# Autodesk Inventor assembly: supports
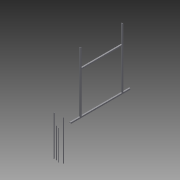
[picture p0: Inventor's stored thumbnail of the model, 180x180]
Saved by Autodesk Inventor 2013 (Build 170138000, 138)
## iProperties
Created: 2012-10-21
Part Number: supports
Document SubType Name: Weldment
Designer: Istvan
Weld Material: Welded Aluminum-6061
Author: Istvan
## Documents named in this file (10)
- D:\GitHub\Crown-Fire\CAD\Frame\Supports\supports.iam
- D:\GitHub\Crown-Fire\CAD\Frame\Supports\leg_bl.ipt
- D:\GitHub\Crown-Fire\CAD\Templates\Angle Iron.ipt
- D:\GitHub\Crown-Fire\CAD\Frame\Supports\leg_br.ipt
- D:\GitHub\Crown-Fire\CAD\Frame\Supports\leg_fl.ipt
- D:\GitHub\Crown-Fire\CAD\Frame\Supports\leg_fr.ipt
- D:\GitHub\Crown-Fire\CAD\Frame\Supports\tableBrace-fb.ipt
- D:\GitHub\Crown-Fire\CAD\Templates\squareTube_1.5.ipt
- D:\GitHub\Crown-Fire\CAD\Frame\Supports\tableBrace-r.ipt
- D:\GitHub\Crown-Fire\CAD\Frame\Supports\tableBrace-l.ipt
## Components (8 placed, 7 different names)
1. leg_bl:1
2. leg_br:2
3. leg_fl:3
4. leg_fr:4
5. tableBrace-fb:1 — Mate:1, Flush:1, Mate:4
6. tableBrace-fb:2 — Mate:2, Flush:2, Mate:3, Flush:3
7. tableBrace-r:3 — Mate:1, Flush:1, Mate:2, Flush:2, Mate:5
8. tableBrace-l:4 — Mate:3, Mate:4, Flush:3, Mate:5
## Relationships (8: Mate 5, Flush 3)
- Mate:1: tableBrace-fb:1 ↔ tableBrace-r:3
- Flush:1: tableBrace-fb:1 ↔ tableBrace-r:3
- Mate:2: tableBrace-fb:2 ↔ tableBrace-r:3
- Flush:2: tableBrace-fb:2 ↔ tableBrace-r:3
- Mate:3: tableBrace-fb:2 ↔ tableBrace-l:4
- Mate:4: tableBrace-fb:1 ↔ tableBrace-l:4
- Flush:3: tableBrace-fb:2 ↔ tableBrace-l:4
- Mate:5 (1244.6 mm): tableBrace-r:3 ↔ tableBrace-l:4
